# Autodesk Inventor assembly: fuse holder
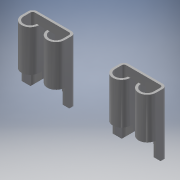
[picture p0: Inventor's stored thumbnail of the model, 180x180]
Saved by Autodesk Inventor 2019.3 (Build 233278000, 278)
## iProperties
Created: 2019-11-25
Part Number: fuse holder
Document SubType Name: Assembly
Designer: kjdix
Author: kjdix
## Documents named in this file (2)
- C:\Users\kjdix\Documents\EAGLE\projects\BLDC-v1\Design files\drv8353 bldc\component models\fuse holder.iam
- C:\Users\kjdix\Documents\EAGLE\projects\BLDC-v1\Design files\drv8353 bldc\component models\fuse clip.ipt
## Components (2 placed, 1 different names)
1. fuse clip:1 — Flush:1, Flush:2, Flush:3, Flush:4, Flush:5, Flush:6
2. fuse clip:2 — Flush:1, Flush:2, Flush:3
## Relationships (6: Flush 6)
- Flush:1: fuse clip:1 ↔ fuse clip:2
- Flush:2: fuse clip:1 ↔ fuse clip:2
- Flush:3 (21.0312 mm): fuse clip:1 ↔ fuse clip:2
- Flush:4: fuse clip:1
- Flush:5 (5.5372 mm): fuse clip:1
- Flush:6: fuse clip:1
